# Autodesk Inventor assembly: ASSY_TREBUCHET_DESIGN2
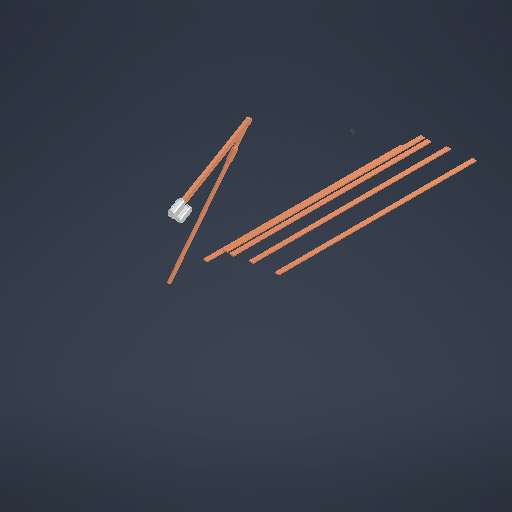
[picture p0: Inventor's stored thumbnail of the model, 512x512]
Saved by Autodesk Inventor 2026.2 (Build 302298010, 298A)
## iProperties
Created: 2026-02-10
Part Number: ASSY_TREBUCHET_DESIGN2
Document SubType Name: Assembly
Designer: 4aida
Author: 4aida
## Documents named in this file (9)
- C:\Users\4aida\OneDrive\Documents\GitHub\Design_II_Group6\Trebuchet\WIPPER_TREBUCHET\ASSY_TREBUCHET_DESIGN2.iam
- C:\Users\4aida\OneDrive\Documents\GitHub\Design_II_Group6\Trebuchet\Canette-355ml.ipt
- C:\Users\4aida\OneDrive\Documents\GitHub\Design_II_Group6\Trebuchet\DOWEL_STOCK_TREBUCHET.ipt
- C:\Users\4aida\OneDrive\Documents\GitHub\Design_II_Group6\Trebuchet\WOOD_STOCK_TREBUCHET.ipt
- C:\Users\4aida\OneDrive\Documents\GitHub\Design_II_Group6\Trebuchet\Yellow_dot_squash_ball,Trebuchet.ipt
- C:\Users\4aida\OneDrive\Documents\GitHub\Design_II_Group6\Trebuchet\WIPPER_TREBUCHET\wipper_arm.ipt
- C:\Users\4aida\OneDrive\Documents\GitHub\Design_II_Group6\Trebuchet\COUNTERWEIGHT_INSIDE_ARM,TREBUCHET.ipt
- C:\Users\4aida\OneDrive\Documents\GitHub\Design_II_Group6\Trebuchet\COUNTERWEIGHT_OUTSIDE_ARM,TREBUCHET.ipt
- C:\Users\4aida\OneDrive\Documents\GitHub\Design_II_Group6\Trebuchet\PIVOT_SPACERS,TREBUCHET.ipt
## Components (16 placed, 8 different names)
1. Canette-355ml:1 — Tangent:1, Tangent:2, Flush:1, Flush:2
2. DOWEL_STOCK_TREBUCHET:1
3. WOOD_STOCK_TREBUCHET:1
4. Yellow_dot_squash_ball,Trebuchet:1
5. Canette-355ml:2 — Tangent:2, Tangent:3, Flush:2
6. Canette-355ml:3 — Tangent:1, Tangent:3, Flush:1, Mate:7
7. WOOD_STOCK_TREBUCHET:2
8. WOOD_STOCK_TREBUCHET:3
9. WOOD_STOCK_TREBUCHET:4
10. WOOD_STOCK_TREBUCHET:5
11. wipper_arm:1 — Mate:1, Mate:2, Flush:3, Mate:3, Mate:4, Mate:6, Mate:8, Mate:9, Mate:10, Mate:11, Flush:7, Flush:8
12. COUNTERWEIGHT_INSIDE_ARM,TREBUCHET:1 — Flush:3, Flush:4, Flush:5, Flush:6, Mate:7
13. COUNTERWEIGHT_OUTSIDE_ARM,TREBUCHET:1 — Mate:3, Mate:5, Mate:6, Flush:5
14. COUNTERWEIGHT_OUTSIDE_ARM,TREBUCHET:2 — Mate:4, Mate:5, Flush:4, Flush:6
15. PIVOT_SPACERS,TREBUCHET:1 — Mate:9, Mate:10, Flush:8
16. PIVOT_SPACERS,TREBUCHET:2 — Mate:8, Mate:11, Flush:7
## Relationships (22: Mate 11, Flush 8, Tangent 3)
- Tangent:1: Canette-355ml:1 ↔ Canette-355ml:3
- Tangent:2: Canette-355ml:1 ↔ Canette-355ml:2
- Tangent:3: Canette-355ml:2 ↔ Canette-355ml:3
- Flush:1: Canette-355ml:1 ↔ Canette-355ml:3
- Flush:2: Canette-355ml:1 ↔ Canette-355ml:2
- Mate:1: wipper_arm:1
- Mate:2: wipper_arm:1
- Flush:3: wipper_arm:1 ↔ COUNTERWEIGHT_INSIDE_ARM,TREBUCHET:1
- Mate:3: wipper_arm:1 ↔ COUNTERWEIGHT_OUTSIDE_ARM,TREBUCHET:1
- Mate:4: wipper_arm:1 ↔ COUNTERWEIGHT_OUTSIDE_ARM,TREBUCHET:2
- Mate:5: COUNTERWEIGHT_OUTSIDE_ARM,TREBUCHET:1 ↔ COUNTERWEIGHT_OUTSIDE_ARM,TREBUCHET:2
- Mate:6: wipper_arm:1 ↔ COUNTERWEIGHT_OUTSIDE_ARM,TREBUCHET:1
- Flush:4: COUNTERWEIGHT_INSIDE_ARM,TREBUCHET:1 ↔ COUNTERWEIGHT_OUTSIDE_ARM,TREBUCHET:2
- Flush:5: COUNTERWEIGHT_INSIDE_ARM,TREBUCHET:1 ↔ COUNTERWEIGHT_OUTSIDE_ARM,TREBUCHET:1
- Flush:6: COUNTERWEIGHT_INSIDE_ARM,TREBUCHET:1 ↔ COUNTERWEIGHT_OUTSIDE_ARM,TREBUCHET:2
- Mate:7: Canette-355ml:3 ↔ COUNTERWEIGHT_INSIDE_ARM,TREBUCHET:1
- Mate:8: wipper_arm:1 ↔ PIVOT_SPACERS,TREBUCHET:2
- Mate:9: wipper_arm:1 ↔ PIVOT_SPACERS,TREBUCHET:1
- Mate:10: wipper_arm:1 ↔ PIVOT_SPACERS,TREBUCHET:1
- Mate:11: wipper_arm:1 ↔ PIVOT_SPACERS,TREBUCHET:2
- Flush:7: wipper_arm:1 ↔ PIVOT_SPACERS,TREBUCHET:2
- Flush:8: wipper_arm:1 ↔ PIVOT_SPACERS,TREBUCHET:1
